# Autodesk Inventor assembly: Chassis Assembly
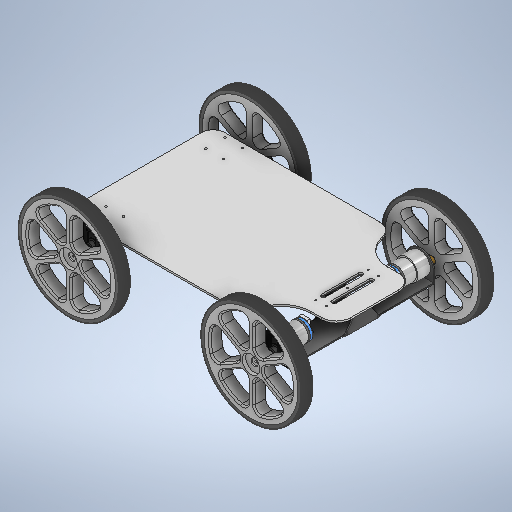
[picture p0: Inventor's stored thumbnail of the model, 512x512]
Saved by Autodesk Inventor 2025.2 (Build 292293000, 293)
## iProperties
Created: 2025-01-16
Part Number: Chassis Assembly
Document SubType Name: Assembly
Designer: Matt Tidd
Author: Matt Tidd
## Documents named in this file (5)
- C:\Users\mtidd2\Desktop\H2A\CAD\Chassis_Design\Chassis Assembly.iam
- C:\Users\mtidd2\Desktop\H2A\CAD\Motors_and_Wheels\Pendulum Suspension\Pendulum Suspension Assembly.iam
- C:\Users\mtidd2\Desktop\H2A\CAD\Chassis_Design\Chassis Bottom Plate.ipt
- C:\Users\mtidd2\Desktop\H2A\CAD\Motors_and_Wheels\Wheel Assembly\Motor Wheel Assembly.iam
- C:\Users\mtidd2\Desktop\H2A\CAD\TrashStorageUnit\Garbage Can Mockup.ipt
## Components (5 placed, 4 different names)
1. Pendulum Suspension Assembly:1 [sub-assembly] — Mate:1
2. Chassis Bottom Plate:1 — Mate:1, Mate:2, Mate:3, Mate:4, Mate:5, Mate:6, Mate:7
3. Motor Wheel Assembly:1 [sub-assembly] — Mate:2, Mate:3
4. Motor Wheel Assembly:2 [sub-assembly] — Mate:4, Mate:5
5. Garbage Can Mockup:1 — Mate:6, Mate:7
## Relationships (7: Mate 7)
- Mate:1: Pendulum Suspension Assembly:1 ↔ Chassis Bottom Plate:1
- Mate:2: Chassis Bottom Plate:1 ↔ Motor Wheel Assembly:1
- Mate:3: Chassis Bottom Plate:1 ↔ Motor Wheel Assembly:1
- Mate:4: Chassis Bottom Plate:1 ↔ Motor Wheel Assembly:2
- Mate:5: Chassis Bottom Plate:1 ↔ Motor Wheel Assembly:2
- Mate:6: Chassis Bottom Plate:1 ↔ Garbage Can Mockup:1
- Mate:7: Chassis Bottom Plate:1 ↔ Garbage Can Mockup:1
